# Autodesk Inventor assembly: E3DV6
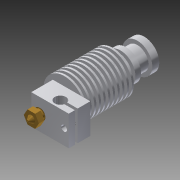
[picture p0: Inventor's stored thumbnail of the model, 180x180]
Saved by Autodesk Inventor 2015 (Build 190159000, 159)
## iProperties
Created: 2014-08-17
Part Number: E3DV6
Document SubType Name: Assembly
Designer: Jack
Author: Jack
## Documents named in this file (5)
- C:\Users\Jack\ownCloud\Projects\CoreXY\InventorModel\HotEnds\E3DV6\E3DV6.iam
- C:\Users\Jack\ownCloud\Projects\CoreXY\InventorModel\HotEnds\E3DV6\E3DV6HeatBreak.ipt
- C:\Users\Jack\ownCloud\Projects\CoreXY\InventorModel\HotEnds\E3DV6\E3DV6HeatSink.ipt
- C:\Users\Jack\ownCloud\Projects\CoreXY\InventorModel\HotEnds\E3DV6\E3DV6Nozzle.ipt
- C:\Users\Jack\ownCloud\Projects\CoreXY\InventorModel\HotEnds\E3DV6\E3DV6NozzleBlock.ipt
## Components (4 placed, 4 different names)
1. E3DV6HeatBreak:1 — Mate:1, Mate:2, Mate:3, Mate:5
2. E3DV6HeatSink:1 — Mate:1, Mate:2
3. E3DV6Nozzle:1 — Mate:4, Mate:5, Flush:1
4. E3DV6NozzleBlock:1 — Mate:3, Mate:4, Flush:1
## Relationships (6: Mate 5, Flush 1)
- Mate:1: E3DV6HeatBreak:1 ↔ E3DV6HeatSink:1
- Mate:2: E3DV6HeatBreak:1 ↔ E3DV6HeatSink:1
- Mate:3: E3DV6HeatBreak:1 ↔ E3DV6NozzleBlock:1
- Mate:4: E3DV6Nozzle:1 ↔ E3DV6NozzleBlock:1
- Mate:5: E3DV6HeatBreak:1 ↔ E3DV6Nozzle:1
- Flush:1: E3DV6Nozzle:1 ↔ E3DV6NozzleBlock:1
